# Autodesk Inventor assembly: GateAssembly
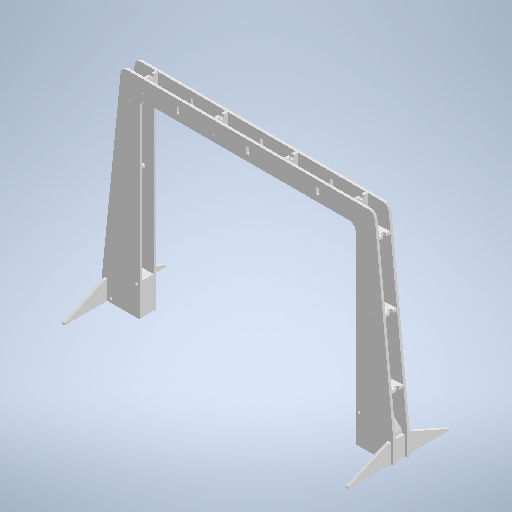
[picture p0: Inventor's stored thumbnail of the model, 512x512]
Saved by Autodesk Inventor 2025.1 (Build 291241000, 241)
## iProperties
Created: 2025-03-30
Part Number: GateAssembly
Document SubType Name: Assembly
Designer: 42060
Author: 42060
## Documents named in this file (5)
- C:\Users\42060\Desktop\School\Projects\RoboClash\LineFollower_Gate\GateAssembly.iam
- C:\Users\42060\Desktop\School\Projects\RoboClash\LineFollower_Gate\GateBrigeSide.ipt
- C:\Users\42060\Desktop\School\Projects\RoboClash\LineFollower_Gate\Leg.ipt
- C:\Users\42060\Desktop\School\Projects\RoboClash\LineFollower_Gate\Sensor.ipt
- C:\Users\42060\Desktop\School\Projects\RoboClash\LineFollower_Gate\Spacer.ipt
## Components (16 placed, 4 different names)
1. GateBrigeSide:1 — Vložit:1, Vložit:2, Vložit:3, Vložit:4, Proti sobě:1, Proti sobě:6, Proti sobě:7, Stejný směr:2, Proti sobě:8, Proti sobě:9, Stejný směr:3, Stejný směr:4, Stejný směr:5, Proti sobě:10, Stejný směr:7, Proti sobě:11, Proti sobě:12, Stejný směr:8, Proti sobě:13, Stejný směr:9, Stejný směr:10, Proti sobě:14, Stejný směr:11, Stejný směr:12, Proti sobě:15, Stejný směr:13, Stejný směr:14, Proti sobě:16, Stejný směr:15, Stejný směr:16, Proti sobě:17, Stejný směr:17, Stejný směr:18, Proti sobě:18
2. Leg:1 — Proti sobě:1, Proti sobě:2, Proti sobě:3
3. Sensor:1 — Vložit:1, Vložit:2, Vložit:5
4. Spacer:1 — Proti sobě:7, Stejný směr:1, Stejný směr:2
5. Sensor:2 — Vložit:3, Vložit:4, Vložit:6
6. GateBrigeSide:2 — Vložit:5, Vložit:6, Proti sobě:2, Proti sobě:3, Proti sobě:4, Proti sobě:5, Stejný směr:1, Stejný směr:6
7. Leg:2 — Proti sobě:4, Proti sobě:5, Proti sobě:6
8. Spacer:2 — Proti sobě:8, Proti sobě:9, Stejný směr:3
9. Spacer:3 — Stejný směr:4, Stejný směr:5, Proti sobě:10
10. Spacer:4 — Stejný směr:6, Stejný směr:7, Proti sobě:11
11. Spacer:5 — Proti sobě:12, Stejný směr:8, Proti sobě:13
12. Spacer:6 — Stejný směr:9, Stejný směr:10, Proti sobě:14
13. Spacer:7 — Stejný směr:17, Stejný směr:18, Proti sobě:18
14. Spacer:8 — Stejný směr:15, Stejný směr:16, Proti sobě:17
15. Spacer:9 — Stejný směr:13, Stejný směr:14, Proti sobě:16
16. Spacer:10 — Stejný směr:11, Stejný směr:12, Proti sobě:15
## Relationships (42: Mate 18, Flush 18, Insert 6)
- Vložit:1 [Insert]: GateBrigeSide:1 ↔ Sensor:1
- Vložit:2 [Insert]: GateBrigeSide:1 ↔ Sensor:1
- Vložit:3 [Insert]: GateBrigeSide:1 ↔ Sensor:2
- Vložit:4 [Insert]: GateBrigeSide:1 ↔ Sensor:2
- Vložit:5 [Insert]: Sensor:1 ↔ GateBrigeSide:2
- Vložit:6 [Insert]: Sensor:2 ↔ GateBrigeSide:2
- Proti sobě:1 [Mate]: GateBrigeSide:1 ↔ Leg:1
- Proti sobě:2 [Mate]: Leg:1 ↔ GateBrigeSide:2
- Proti sobě:3 [Mate]: Leg:1 ↔ GateBrigeSide:2
- Proti sobě:4 [Mate]: GateBrigeSide:2 ↔ Leg:2
- Proti sobě:5 [Mate]: GateBrigeSide:2 ↔ Leg:2
- Proti sobě:6 [Mate]: GateBrigeSide:1 ↔ Leg:2
- Proti sobě:7 [Mate]: GateBrigeSide:1 ↔ Spacer:1
- Stejný směr:1 [Flush]: Spacer:1 ↔ GateBrigeSide:2
- Stejný směr:2 [Flush] (0.1 mm): GateBrigeSide:1 ↔ Spacer:1
- Proti sobě:8 [Mate]: GateBrigeSide:1 ↔ Spacer:2
- Proti sobě:9 [Mate]: GateBrigeSide:1 ↔ Spacer:2
- Stejný směr:3 [Flush] (0.1 mm): GateBrigeSide:1 ↔ Spacer:2
- Stejný směr:4 [Flush]: GateBrigeSide:1 ↔ Spacer:3
- Stejný směr:5 [Flush] (0.1 mm): GateBrigeSide:1 ↔ Spacer:3
- Proti sobě:10 [Mate]: GateBrigeSide:1 ↔ Spacer:3
- Stejný směr:6 [Flush]: GateBrigeSide:2 ↔ Spacer:4
- Stejný směr:7 [Flush] (0.1 mm): GateBrigeSide:1 ↔ Spacer:4
- Proti sobě:11 [Mate]: GateBrigeSide:1 ↔ Spacer:4
- Proti sobě:12 [Mate]: GateBrigeSide:1 ↔ Spacer:5
- Stejný směr:8 [Flush] (0.1 mm): GateBrigeSide:1 ↔ Spacer:5
- Proti sobě:13 [Mate]: GateBrigeSide:1 ↔ Spacer:5
- Stejný směr:9 [Flush]: GateBrigeSide:1 ↔ Spacer:6
- Stejný směr:10 [Flush] (0.1 mm): GateBrigeSide:1 ↔ Spacer:6
- Proti sobě:14 [Mate]: GateBrigeSide:1 ↔ Spacer:6
- Stejný směr:11 [Flush]: GateBrigeSide:1 ↔ Spacer:10
- Stejný směr:12 [Flush] (0.1 mm): GateBrigeSide:1 ↔ Spacer:10
- Proti sobě:15 [Mate]: GateBrigeSide:1 ↔ Spacer:10
- Stejný směr:13 [Flush]: GateBrigeSide:1 ↔ Spacer:9
- Stejný směr:14 [Flush] (0.1 mm): GateBrigeSide:1 ↔ Spacer:9
- Proti sobě:16 [Mate]: GateBrigeSide:1 ↔ Spacer:9
- Stejný směr:15 [Flush]: GateBrigeSide:1 ↔ Spacer:8
- Stejný směr:16 [Flush] (0.1 mm): GateBrigeSide:1 ↔ Spacer:8
- Proti sobě:17 [Mate]: GateBrigeSide:1 ↔ Spacer:8
- Stejný směr:17 [Flush]: GateBrigeSide:1 ↔ Spacer:7
- Stejný směr:18 [Flush] (0.1 mm): GateBrigeSide:1 ↔ Spacer:7
- Proti sobě:18 [Mate]: GateBrigeSide:1 ↔ Spacer:7
